# Autodesk Inventor assembly: Delts Robot V1 Assembly
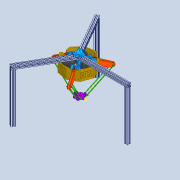
[picture p0: Inventor's stored thumbnail of the model, 180x180]
Saved by Autodesk Inventor 2022 (Build 260153000, 153)
## iProperties
Created: 2021-03-06
Part Number: Delts Robot V1 Assembly
Document SubType Name: Assembly
Designer: Coy
Author: Coy
## Documents named in this file (10)
- H:\3D Files\Project 3D Models\Delta Robot\Delts Robot V1 Assembly.iam
- H:\3D Files\Project 3D Models\Delta Robot\Delts Robot Motor Hub.ipt
- H:\3D Files\Project 3D Models\Delta Robot\Nema 17 CNC Kit Stepper Motor.ipt
- H:\3D Files\Project 3D Models\Delta Robot\Delta Robot Arm Segment One.ipt
- H:\3D Files\Project 3D Models\Delta Robot\Delta Robot Arm Segment Two.ipt
- H:\3D Files\Project 3D Models\Delta Robot\Delts Robot Cairage.ipt
- H:\3D Files\Project 3D Models\Delta Robot\Delts Robot Arm Joint Rod.ipt
- H:\3D Files\Project 3D Models\Delta Robot\2020-aluminium-profile-v-slot-solidwork2016-1.snapshot.8\2020 aluminium profile v slot solidwork2016.ipt
- H:\3D Files\Project 3D Models\Delta Robot\Small GT2 Belt Pully.ipt
- H:\3D Files\Project 3D Models\Delta Robot\Delta Robot Siding Piece.ipt
## Components (30 placed, 9 different names)
1. Delts Robot Motor Hub:1 — Mate:1, Flush:1, Mate:3, Flush:2, Flush:3, Mate:7, Mate:8, Mate:9, Mate:10, Mate:11, Mate:12, Angle:1, Mate:20, Mate:22, Mate:25, Mate:28, Mate:32, Angle:3, Angle:4, Angle:5, Mate:35, Mate:36, Mate:39, Mate:40, Mate:41, Mate:42
2. Nema 17 CNC Kit Stepper Motor:1 — Flush:3, Mate:32, Angle:3
3. Nema 17 CNC Kit Stepper Motor:2 — Mate:3, Flush:2, Angle:5, Mate:33, Mate:34
4. Nema 17 CNC Kit Stepper Motor:3 — Mate:1, Flush:1, Angle:4
5. Delta Robot Arm Segment One:1 — Mate:7, Mate:8, Mate:13, Flush:4
6. Delta Robot Arm Segment One:2 — Mate:11, Mate:12, Mate:17, Flush:8
7. Delta Robot Arm Segment One:3 — Mate:9, Mate:10, Mate:18, Flush:9
8. Delta Robot Arm Segment Two:1 — Ball:1, Ball:11
9. Delta Robot Arm Segment Two:2 — Ball:2, Ball:12
10. Delta Robot Arm Segment Two:3 — Ball:6, Ball:7
11. Delta Robot Arm Segment Two:4 — Ball:5, Ball:8
12. Delta Robot Arm Segment Two:5 — Ball:4, Ball:9
13. Delta Robot Arm Segment Two:6 — Ball:3, Ball:10
14. Delts Robot Cairage:1 — Mate:14, Flush:5, Mate:15, Flush:6, Mate:16, Flush:7, Angle:1
15. Delts Robot Arm Joint Rod:1 — Mate:13, Flush:4, Ball:1, Ball:2
16. Delts Robot Arm Joint Rod:2 — Mate:14, Flush:5, Ball:11, Ball:12
17. Delts Robot Arm Joint Rod:3 — Mate:16, Flush:7, Ball:7, Ball:8
18. Delts Robot Arm Joint Rod:4 — Mate:15, Flush:6, Ball:9, Ball:10
19. Delts Robot Arm Joint Rod:5 — Mate:17, Flush:8, Ball:3, Ball:4
20. Delts Robot Arm Joint Rod:6 — Mate:18, Flush:9, Ball:5, Ball:6
21. 2020 aluminium profile v slot solidwork2016:1 — Mate:20, Mate:28, Flush:11, Flush:12, Mate:29
22. 2020 aluminium profile v slot solidwork2016:2 — Mate:25, Flush:15, Flush:16, Mate:31
23. 2020 aluminium profile v slot solidwork2016:3 — Mate:22, Flush:13, Flush:14, Mate:30
24. 2020 aluminium profile v slot solidwork2016:4 — Flush:11, Flush:12, Mate:29
25. 2020 aluminium profile v slot solidwork2016:5 — Flush:13, Flush:14, Mate:30
26. 2020 aluminium profile v slot solidwork2016:6 — Flush:15, Flush:16, Mate:31
27. Small GT2 Belt Pully:1 — Mate:33, Mate:34
28. Delta Robot Siding Piece:1 — Mate:35, Mate:36
29. Delta Robot Siding Piece:3 — Mate:39, Mate:40
30. Delta Robot Siding Piece:4 — Mate:41, Mate:42
## Relationships (61: Mate 30, Flush 15, BallJoint 12, Angle 4)
- Mate:1: Delts Robot Motor Hub:1 ↔ Nema 17 CNC Kit Stepper Motor:3
- Flush:1 (4 mm): Delts Robot Motor Hub:1 ↔ Nema 17 CNC Kit Stepper Motor:3
- Mate:3: Delts Robot Motor Hub:1 ↔ Nema 17 CNC Kit Stepper Motor:2
- Flush:2 (4 mm): Delts Robot Motor Hub:1 ↔ Nema 17 CNC Kit Stepper Motor:2
- Flush:3 (4 mm): Delts Robot Motor Hub:1 ↔ Nema 17 CNC Kit Stepper Motor:1
- Mate:7: Delts Robot Motor Hub:1 ↔ Delta Robot Arm Segment One:1
- Mate:8 (1 mm): Delts Robot Motor Hub:1 ↔ Delta Robot Arm Segment One:1
- Mate:9: Delts Robot Motor Hub:1 ↔ Delta Robot Arm Segment One:3
- Mate:10 (1 mm): Delts Robot Motor Hub:1 ↔ Delta Robot Arm Segment One:3
- Mate:11: Delts Robot Motor Hub:1 ↔ Delta Robot Arm Segment One:2
- Mate:12 (1 mm): Delts Robot Motor Hub:1 ↔ Delta Robot Arm Segment One:2
- Mate:13: Delta Robot Arm Segment One:1 ↔ Delts Robot Arm Joint Rod:1
- Flush:4 (-7.5 mm): Delta Robot Arm Segment One:1 ↔ Delts Robot Arm Joint Rod:1
- Ball:1: Delta Robot Arm Segment Two:1 ↔ Delts Robot Arm Joint Rod:1
- Ball:2: Delta Robot Arm Segment Two:2 ↔ Delts Robot Arm Joint Rod:1
- Mate:14: Delts Robot Cairage:1 ↔ Delts Robot Arm Joint Rod:2
- Flush:5 (-7.5 mm): Delts Robot Cairage:1 ↔ Delts Robot Arm Joint Rod:2
- Mate:15: Delts Robot Cairage:1 ↔ Delts Robot Arm Joint Rod:4
- Flush:6 (-7.5 mm): Delts Robot Cairage:1 ↔ Delts Robot Arm Joint Rod:4
- Mate:16: Delts Robot Cairage:1 ↔ Delts Robot Arm Joint Rod:3
- Flush:7 (-7.5 mm): Delts Robot Cairage:1 ↔ Delts Robot Arm Joint Rod:3
- Mate:17: Delta Robot Arm Segment One:2 ↔ Delts Robot Arm Joint Rod:5
- Flush:8 (-7.5 mm): Delta Robot Arm Segment One:2 ↔ Delts Robot Arm Joint Rod:5
- Mate:18: Delta Robot Arm Segment One:3 ↔ Delts Robot Arm Joint Rod:6
- Flush:9 (-7.5 mm): Delta Robot Arm Segment One:3 ↔ Delts Robot Arm Joint Rod:6
- Ball:3: Delta Robot Arm Segment Two:6 ↔ Delts Robot Arm Joint Rod:5
- Ball:4: Delta Robot Arm Segment Two:5 ↔ Delts Robot Arm Joint Rod:5
- Ball:5: Delta Robot Arm Segment Two:4 ↔ Delts Robot Arm Joint Rod:6
- Ball:6: Delta Robot Arm Segment Two:3 ↔ Delts Robot Arm Joint Rod:6
- Ball:7: Delta Robot Arm Segment Two:3 ↔ Delts Robot Arm Joint Rod:3
- Ball:8: Delta Robot Arm Segment Two:4 ↔ Delts Robot Arm Joint Rod:3
- Ball:9: Delta Robot Arm Segment Two:5 ↔ Delts Robot Arm Joint Rod:4
- Ball:10: Delta Robot Arm Segment Two:6 ↔ Delts Robot Arm Joint Rod:4
- Ball:11: Delta Robot Arm Segment Two:1 ↔ Delts Robot Arm Joint Rod:2
- Angle:1 (0 deg): Delts Robot Motor Hub:1 ↔ Delts Robot Cairage:1
- Ball:12: Delta Robot Arm Segment Two:2 ↔ Delts Robot Arm Joint Rod:2
- Mate:20: Delts Robot Motor Hub:1 ↔ 2020 aluminium profile v slot solidwork2016:1
- Mate:22: Delts Robot Motor Hub:1 ↔ 2020 aluminium profile v slot solidwork2016:3
- Mate:25: Delts Robot Motor Hub:1 ↔ 2020 aluminium profile v slot solidwork2016:2
- Mate:28: Delts Robot Motor Hub:1 ↔ 2020 aluminium profile v slot solidwork2016:1
- Flush:11: 2020 aluminium profile v slot solidwork2016:1 ↔ 2020 aluminium profile v slot solidwork2016:4
- Flush:12: 2020 aluminium profile v slot solidwork2016:1 ↔ 2020 aluminium profile v slot solidwork2016:4
- Mate:29: 2020 aluminium profile v slot solidwork2016:1 ↔ 2020 aluminium profile v slot solidwork2016:4
- Flush:13: 2020 aluminium profile v slot solidwork2016:3 ↔ 2020 aluminium profile v slot solidwork2016:5
- Flush:14: 2020 aluminium profile v slot solidwork2016:3 ↔ 2020 aluminium profile v slot solidwork2016:5
- Mate:30: 2020 aluminium profile v slot solidwork2016:3 ↔ 2020 aluminium profile v slot solidwork2016:5
- Flush:15: 2020 aluminium profile v slot solidwork2016:2 ↔ 2020 aluminium profile v slot solidwork2016:6
- Flush:16: 2020 aluminium profile v slot solidwork2016:2 ↔ 2020 aluminium profile v slot solidwork2016:6
- Mate:31: 2020 aluminium profile v slot solidwork2016:2 ↔ 2020 aluminium profile v slot solidwork2016:6
- Mate:32: Delts Robot Motor Hub:1 ↔ Nema 17 CNC Kit Stepper Motor:1
- Angle:3 (0 deg): Delts Robot Motor Hub:1 ↔ Nema 17 CNC Kit Stepper Motor:1
- Angle:4 (0 deg): Delts Robot Motor Hub:1 ↔ Nema 17 CNC Kit Stepper Motor:3
- Angle:5 (0 deg): Delts Robot Motor Hub:1 ↔ Nema 17 CNC Kit Stepper Motor:2
- Mate:33: Nema 17 CNC Kit Stepper Motor:2 ↔ Small GT2 Belt Pully:1
- Mate:34 (0.5 mm): Nema 17 CNC Kit Stepper Motor:2 ↔ Small GT2 Belt Pully:1
- Mate:35: Delts Robot Motor Hub:1 ↔ Delta Robot Siding Piece:1
- Mate:36: Delts Robot Motor Hub:1 ↔ Delta Robot Siding Piece:1
- Mate:39: Delts Robot Motor Hub:1 ↔ Delta Robot Siding Piece:3
- Mate:40: Delts Robot Motor Hub:1 ↔ Delta Robot Siding Piece:3
- Mate:41: Delts Robot Motor Hub:1 ↔ Delta Robot Siding Piece:4
- Mate:42: Delts Robot Motor Hub:1 ↔ Delta Robot Siding Piece:4
